# Autodesk Inventor assembly: gusset_back
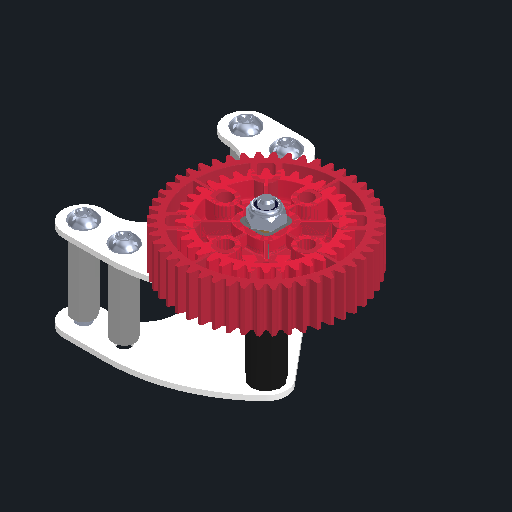
[picture p0: Inventor's stored thumbnail of the model, 512x512]
Saved by Autodesk Inventor 2025 (Build 290162000, 162)
## iProperties
Created: 2024-08-21
Part Number: gusset_back
Document SubType Name: Assembly
Designer: averey
Author: averey
## Documents named in this file (7)
- D:\vex_robotics_high_stakes\hardware\cad\bots\ENIGMA\chassis\drivetrain\drivebay\gusset_back\gusset_back.iam
- D:\vex_robotics_high_stakes\hardware\cad\bots\ENIGMA\chassis\drivetrain\drivebay\gusset_back\gusset_back.ipt
- D:\vex_robotics_high_stakes\hardware\cad\VEX-CAD-Inventor\Structure\Standoff\Standoff .875.ipt
- D:\vex_robotics_high_stakes\hardware\cad\VEX-CAD-Inventor\Structure\Hardware\Screw Shoulder Robosource\SScrew Shoulder Smooth .290 x .09.ipt
- D:\vex_robotics_high_stakes\hardware\cad\bots\ENIGMA\chassis\drivetrain\drivebay\gusset_back\wall_glides_back.iam
- D:\vex_robotics_high_stakes\hardware\cad\VEX-CAD-Inventor\Structure\Standoff.ipt
- D:\vex_robotics_high_stakes\hardware\cad\VEX-CAD-Inventor\Structure\Hardware\Screw Shoulder Robosource.ipt
## Components (13 placed, 4 different names)
1. gusset_back:1 — Mate:1, Insert:1, Insert:3, Insert:4, Insert:6
2. gusset_back:2 — Mate:1, Insert:1, Insert:5
3. wall_glides_back:1 [sub-assembly] — Insert:6
4. Standoff .875:1 — Insert:3
5. Standoff .875:2
6. Standoff .875:3
7. Standoff .875:4
8. SScrew Shoulder Smooth .290 x .09:1 — Insert:4
9. SScrew Shoulder Smooth .290 x .09:3
10. SScrew Shoulder Smooth .290 x .09:4
11. SScrew Shoulder Smooth .290 x .09:5
12. SScrew Shoulder Smooth .290 x .09:2 — Insert:5
13. SScrew Shoulder Smooth .290 x .09:6
## Component patterns: (4 elements, first: Standoff .875:1), (4 elements, first: SScrew Shoulder Smooth .290 x .09:1), (2 elements, first: SScrew Shoulder Smooth .290 x .09:2)
## Relationships (6: Insert 5, Mate 1)
- Mate:1: gusset_back:1 ↔ gusset_back:2
- Insert:1 (25.4 mm): gusset_back:1 ↔ gusset_back:2
- Insert:3 (1.5875 mm): gusset_back:1 ↔ Standoff .875:1
- Insert:4: gusset_back:1 ↔ SScrew Shoulder Smooth .290 x .09:1
- Insert:5: gusset_back:2 ↔ SScrew Shoulder Smooth .290 x .09:2
- Insert:6: gusset_back:1 ↔ wall_glides_back:1
